# Autodesk Inventor assembly: spool_sub_assem
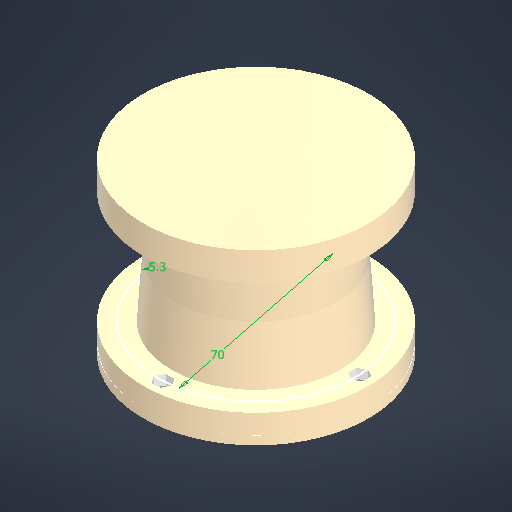
[picture p0: Inventor's stored thumbnail of the model, 512x512]
Saved by Autodesk Inventor 2026.2 (Build 302298010, 298A)
## iProperties
Created: 2026-03-03
Part Number: spool_sub_assem
Document SubType Name: Assembly
Designer: Luke
Author: Luke
## Documents named in this file (5)
- C:\Users\Luke\OneDrive - Heriot-Watt University\Desktop\Robot Mech Sys\GroupProject\CAD\sub_assemblies\spool_sub_assem.iam
- C:\Users\Luke\OneDrive - Heriot-Watt University\Desktop\Robot Mech Sys\GroupProject\CAD\parts\spool.ipt
- C:\Users\Luke\OneDrive - Heriot-Watt University\Desktop\Robot Mech Sys\GroupProject\CAD\parts\spool_motor_side.ipt
- C:\Users\Luke\Documents\Inventor\Content Center Files\R2026\en-US\BS EN ISO 7045 H\EN ISO 7045 - M2 x 6 - 4.8 - H(1).ipt
- C:\Users\Luke\Documents\Inventor\Content Center Files\R2026\en-US\BS EN 24032\ISO 4032 - M2BS EN.ipt
## Components (10 placed, 4 different names)
1. spool:1 — Mate:1, Mate:2, Mate:3, Insert:1, Insert:2, Insert:3, Insert:4
2. spool_motor_side:1 — Mate:1, Mate:2, Mate:3, Mate:12, Mate:13, Mate:14, Mate:15, Mate:16, Mate:17, Mate:18, Mate:19
3. BS EN ISO 7045 H - Metric M2 x 6 - 4.8 - H:1 — Mate:14, Mate:16
4. BS EN ISO 7045 H - Metric M2 x 6 - 4.8 - H:2 — Mate:13, Mate:17
5. BS EN ISO 7045 H - Metric M2 x 6 - 4.8 - H:3 — Mate:15, Mate:19
6. BS EN ISO 7045 H - Metric M2 x 6 - 4.8 - H:4 — Mate:12, Mate:18
7. BS EN 24032 - Metric M2:1 — Insert:1
8. BS EN 24032 - Metric M2:2 — Insert:2
9. BS EN 24032 - Metric M2:3 — Insert:3
10. BS EN 24032 - Metric M2:4 — Insert:4
## Relationships (15: Mate 11, Insert 4)
- Mate:1: spool:1 ↔ spool_motor_side:1
- Mate:2: spool:1 ↔ spool_motor_side:1
- Mate:3: spool:1 ↔ spool_motor_side:1
- Mate:12: spool_motor_side:1 ↔ BS EN ISO 7045 H - Metric M2 x 6 - 4.8 - H:4
- Mate:13: spool_motor_side:1 ↔ BS EN ISO 7045 H - Metric M2 x 6 - 4.8 - H:2
- Mate:14: spool_motor_side:1 ↔ BS EN ISO 7045 H - Metric M2 x 6 - 4.8 - H:1
- Mate:15: spool_motor_side:1 ↔ BS EN ISO 7045 H - Metric M2 x 6 - 4.8 - H:3
- Mate:16: spool_motor_side:1 ↔ BS EN ISO 7045 H - Metric M2 x 6 - 4.8 - H:1
- Mate:17: spool_motor_side:1 ↔ BS EN ISO 7045 H - Metric M2 x 6 - 4.8 - H:2
- Mate:18: spool_motor_side:1 ↔ BS EN ISO 7045 H - Metric M2 x 6 - 4.8 - H:4
- Mate:19: spool_motor_side:1 ↔ BS EN ISO 7045 H - Metric M2 x 6 - 4.8 - H:3
- Insert:1: spool:1 ↔ BS EN 24032 - Metric M2:1
- Insert:2: spool:1 ↔ BS EN 24032 - Metric M2:2
- Insert:3: spool:1 ↔ BS EN 24032 - Metric M2:3
- Insert:4: spool:1 ↔ BS EN 24032 - Metric M2:4
